# Autodesk Inventor assembly: eceuil-complet
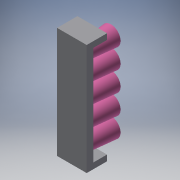
[picture p0: Inventor's stored thumbnail of the model, 180x180]
Saved by Autodesk Inventor 2019 (Build 230136000, 136)
## iProperties
Created: 2020-02-15
Part Number: eceuil-complet
Document SubType Name: Assembly
Designer: franc
Author: franc
## Documents named in this file (3)
- C:\Users\franc\Desktop\EsialRobotik\Mecanique\2020\elements\ecueil-complet.iam
- C:\Users\franc\Desktop\EsialRobotik\Mecanique\2020\elements\ecueil.ipt
- C:\Users\franc\Desktop\EsialRobotik\Mecanique\2020\elements\bouees.ipt
## Components (6 placed, 2 different names)
1. ecueil:1 — Placage:1, Placage:2, Placage:3, Placage:4, Placage:5, Placage:6, Placage:7, Placage:8, Placage:9, Placage:10
2. bouees:1 — Placage:6, Placage:10
3. bouees:2 — Placage:5, Placage:9
4. bouees:3 — Placage:4, Placage:8
5. bouees:4 — Placage:3, Placage:7
6. bouees:5 — Placage:1, Placage:2
## Relationships (10: Mate 10)
- Placage:1 [Mate]: ecueil:1 ↔ bouees:5
- Placage:2 [Mate]: ecueil:1 ↔ bouees:5
- Placage:3 [Mate]: ecueil:1 ↔ bouees:4
- Placage:4 [Mate]: ecueil:1 ↔ bouees:3
- Placage:5 [Mate]: ecueil:1 ↔ bouees:2
- Placage:6 [Mate]: ecueil:1 ↔ bouees:1
- Placage:7 [Mate]: ecueil:1 ↔ bouees:4
- Placage:8 [Mate]: ecueil:1 ↔ bouees:3
- Placage:9 [Mate]: ecueil:1 ↔ bouees:2
- Placage:10 [Mate]: ecueil:1 ↔ bouees:1
